# Autodesk Inventor assembly: assy-3Dprinter
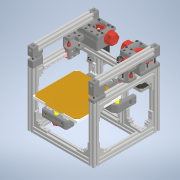
[picture p0: Inventor's stored thumbnail of the model, 180x180]
Saved by Autodesk Inventor 2022 (Build 260153000, 153)
## iProperties
Created: 2021-11-24
Part Number: assy-3Dprinter
Document SubType Name: Assembly
Designer: yuto6
Author: yuto6
## Documents named in this file (4)
- C:\Users\yuto6\Documents\My3DPrinter\CAD\Asm\assy-3Dprinter.iam
- C:\Users\yuto6\Documents\My3DPrinter\CAD\Asm\Frame.iam
- C:\Users\yuto6\Documents\My3DPrinter\CAD\Asm\Z_Bed.iam
- C:\Users\yuto6\Documents\My3DPrinter\CAD\Asm\Gantry.iam
## Components (3 placed, 3 different names)
1. Frame:1 [sub-assembly] — フラッシュ:1, フラッシュ:2, メイト:3, メイト:4, メイト:5
2. Z_Bed:1 [sub-assembly] — メイト:4, メイト:5
3. Gantry:1 [sub-assembly] — フラッシュ:1, フラッシュ:2, メイト:3
## Relationships (5: Mate 3, Flush 2)
- フラッシュ:1 [Flush]: Frame:1 ↔ Gantry:1
- フラッシュ:2 [Flush]: Frame:1 ↔ Gantry:1
- メイト:3 [Mate]: Frame:1 ↔ Gantry:1
- メイト:4 [Mate]: Frame:1 ↔ Z_Bed:1
- メイト:5 [Mate]: Frame:1 ↔ Z_Bed:1
